# Autodesk Inventor assembly: arm_assembly
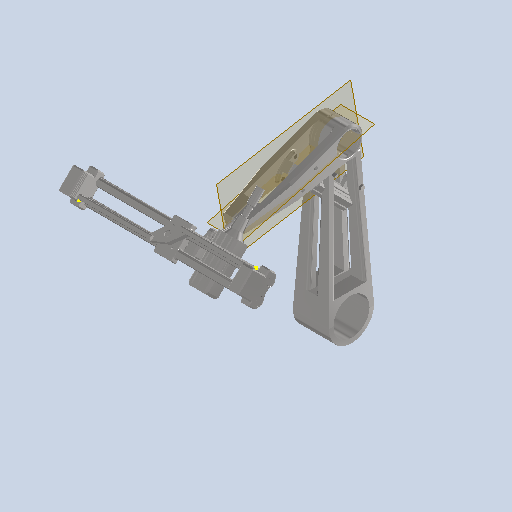
[picture p0: Inventor's stored thumbnail of the model, 512x512]
Saved by Autodesk Inventor 2023 (Build 270158000, 158)
## iProperties
Created: 2023-11-21
Part Number: arm_assembly
Document SubType Name: Assembly
Designer: Beatrice
Author: Beatrice
## Documents named in this file (6)
- E:\WORKSPACE_2\wheel_changing_assignment\arm_assembly.iam
- E:\WORKSPACE_2\wheel_changing_assignment\arm_hydraulic_cylinder.ipt
- E:\WORKSPACE_2\wheel_changing_assignment\robotic_arm_part_3.ipt
- E:\WORKSPACE_2\wheel_changing_assignment\robo_arm_3.1.ipt
- E:\WORKSPACE_2\wheel_changing_assignment\tool_arm_screw.ipt
- E:\WORKSPACE_2\wheel_changing_assignment\clamp_mechanism.iam
## Components (5 placed, 5 different names)
1. arm_hydraulic_cylinder:1 — Mate:1, Mate:2, Mate:3, Mate:8
2. robotic_arm_part_3:2 — Mate:4, Mate:5, Angle:1, Mate:6, Mate:7, Mate:8, Flush:1
3. robo_arm_3.1:1 — Mate:1, Mate:2, Mate:3, Mate:4, Mate:5, Angle:1
4. tool_arm_screw:1 — Mate:6, Mate:7, Mate:9, Mate:10, Mate:11, Flush:1
5. clamp_mechanism:1 [sub-assembly] — Mate:9, Mate:10, Mate:11
## Relationships (13: Mate 11, Angle 1, Flush 1)
- Mate:1: arm_hydraulic_cylinder:1 ↔ robo_arm_3.1:1
- Mate:2: arm_hydraulic_cylinder:1 ↔ robo_arm_3.1:1
- Mate:3: arm_hydraulic_cylinder:1 ↔ robo_arm_3.1:1
- Mate:4: robotic_arm_part_3:2 ↔ robo_arm_3.1:1
- Mate:5: robotic_arm_part_3:2 ↔ robo_arm_3.1:1
- Angle:1 (75 deg): robotic_arm_part_3:2 ↔ robo_arm_3.1:1
- Mate:6: robotic_arm_part_3:2 ↔ tool_arm_screw:1
- Mate:7: robotic_arm_part_3:2 ↔ tool_arm_screw:1
- Mate:8: arm_hydraulic_cylinder:1 ↔ robotic_arm_part_3:2
- Mate:9: tool_arm_screw:1 ↔ clamp_mechanism:1
- Mate:10: tool_arm_screw:1 ↔ clamp_mechanism:1
- Mate:11: tool_arm_screw:1 ↔ clamp_mechanism:1
- Flush:1 (-0.8 mm): robotic_arm_part_3:2 ↔ tool_arm_screw:1
